# Autodesk Inventor assembly: popcorn masala mixing machine
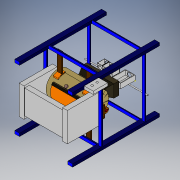
[picture p0: Inventor's stored thumbnail of the model, 180x180]
Saved by Autodesk Inventor 2019 (Build 230136000, 136)
## iProperties
Created: 2019-10-17
Part Number: popcorn masala mixing machine
Document SubType Name: Assembly
Designer: KARTHIK J
Author: KARTHIK J
## Documents named in this file (8)
- C:\Users\KARTHIK J\Documents\popcorn masala mixing machine.iam
- C:\Users\KARTHIK J\Documents\Inventor\17-10-2019.ipt
- C:\Users\KARTHIK J\Documents\stand1111.ipt
- C:\Users\KARTHIK J\Documents\kirans session3.ipt
- C:\Users\KARTHIK J\Documents\kirans session1.ipt
- C:\Users\KARTHIK J\Documents\kirans session2.ipt
- C:\Users\KARTHIK J\Documents\tray final.ipt
- C:\Users\KARTHIK J\Documents\notification.ipt
## Components (10 placed, 7 different names)
1. 17-10-2019:1 — Mate:1
2. stand1111:1
3. stand1111:2
4. kirans session3:2 — Mate:1
5. kirans session1:1
6. kirans session1:2
7. kirans session1:3
8. kirans session2:1
9. tray final:2
10. notification:1
## Relationships (1: Mate 1)
- Mate:1: 17-10-2019:1 ↔ kirans session3:2
